# Autodesk Inventor assembly: Ensamble
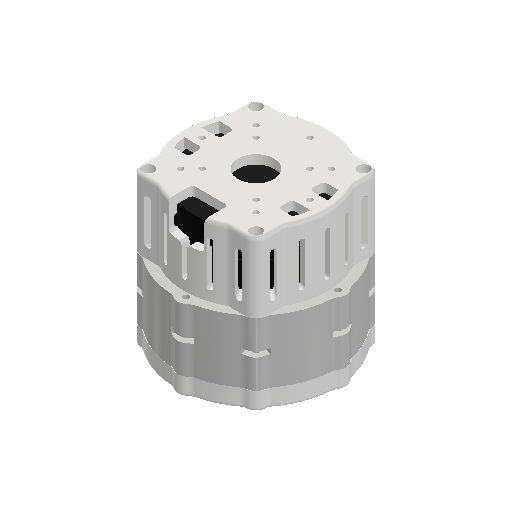
[picture p0: Inventor's stored thumbnail of the model, 512x512]
Saved by Autodesk Inventor 2024.3 (Build 283343000, 343)
## iProperties
Created: 2025-03-05
Part Number: Ensamble
Document SubType Name: Assembly
Designer: danie
Author: danie
## Documents named in this file (8)
- C:\Users\danie\OneDrive\Documentos\Inventor\Motor_drive\Ensamble.iam
- C:\Users\danie\OneDrive\Documentos\Inventor\Motor_drive\motor.ipt
- C:\Users\danie\OneDrive\Documentos\Inventor\Motor_drive\Corona\Corona\Corona.ipt
- C:\Users\danie\OneDrive\Documentos\Inventor\Motor_drive\Portaplanetas.iam
- C:\Users\danie\OneDrive\Documentos\Inventor\Motor_drive\tapa.ipt
- C:\Users\danie\OneDrive\Documentos\Inventor\Motor_drive\adaptador.ipt
- C:\Users\danie\OneDrive\Documentos\Inventor\Motor_drive\Sol\Sol\Sol.ipt
- C:\Users\danie\OneDrive\Documentos\Inventor\Motor_drive\casing.ipt
## Components (7 placed, 7 different names)
1. motor:1 — Mate:1, Flush:1, Mate:2, Mate:4, Mate:5, Mate:7, Mate:8, Mate:9, Mate:10, Mate:16, Mate:17, Mate:21
2. Corona:1 — Mate:5, Mate:15, Mate:18, Mate:19, Mate:20
3. Portaplanetas:1 [sub-assembly] — Mate:4, Mate:14
4. tapa:1 — Mate:7, Mate:15, Mate:20
5. adaptador:1 — Mate:8, Mate:9, Mate:10, Mate:11, Mate:12, Mate:13
6. Sol:1 — Mate:11, Mate:12, Mate:13, Mate:14
7. casing:1 — Mate:16, Mate:17, Mate:18, Mate:19, Mate:21
## Relationships (20: Mate 19, Flush 1)
- Mate:1: motor:1
- Flush:1: motor:1
- Mate:2: motor:1
- Mate:4: motor:1 ↔ Portaplanetas:1
- Mate:5: motor:1 ↔ Corona:1
- Mate:7: motor:1 ↔ tapa:1
- Mate:8: motor:1 ↔ adaptador:1
- Mate:9: motor:1 ↔ adaptador:1
- Mate:10: motor:1 ↔ adaptador:1
- Mate:11: adaptador:1 ↔ Sol:1
- Mate:12: adaptador:1 ↔ Sol:1
- Mate:13: adaptador:1 ↔ Sol:1
- Mate:14: Portaplanetas:1 ↔ Sol:1
- Mate:15: Corona:1 ↔ tapa:1
- Mate:16: motor:1 ↔ casing:1
- Mate:17: motor:1 ↔ casing:1
- Mate:18: Corona:1 ↔ casing:1
- Mate:19: Corona:1 ↔ casing:1
- Mate:20: Corona:1 ↔ tapa:1
- Mate:21: motor:1 ↔ casing:1
